# Autodesk Inventor assembly: Złożenie całości
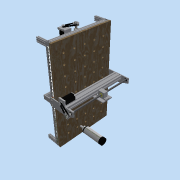
[picture p0: Inventor's stored thumbnail of the model, 180x180]
Saved by Autodesk Inventor 2018 (Build 220112000, 112)
## iProperties
Created: 2019-01-23
Part Number: Złożenie całości
Material: Ogólny
Document SubType Name: Assembly
Designer: Dawid
Author: Dawid
## Documents named in this file (38)
- E:\Frezarka_K2\INVENTOR\ZŁOŻENIA\Złożenie całości.iam
- E:\Frezarka_K2\INVENTOR\RAMA\Profil dolny długi.ipt
- E:\Frezarka_K2\INVENTOR\RAMA\Profil dolny krótki.ipt
- E:\Frezarka_K2\INVENTOR\RAMA\Profil dolny - noga.ipt
- E:\Frezarka_K2\INVENTOR\NAPĘD\Śruba trapezowa 16x4.ipt
- E:\Frezarka_K2\INVENTOR\NAPĘD\Łożysko w obudowie aluminiowej 10mm KP000.ipt
- C:\Users\Dawid\Documents\Inventor\Content Center Files\R2018\pl-PL\DIN 6926\DIN 6926 - M10 x 1,5.ipt
- E:\Frezarka_K2\INVENTOR\NAPĘD\Koło zębate 21 T5 28 2F.ipt
- E:\Frezarka_K2\INVENTOR\NAPĘD\Tuleja zaciskowo rozprężna RCK BK 80 8x15 Clampex.ipt
- C:\Users\Dawid\Documents\Inventor\Content Center Files\R2018\pl-PL\CNS 3932\CNS 3932 - M 4 x 0,7 x 6.ipt
- E:\Frezarka_K2\INVENTOR\NAPĘD\Silnik krokowy SM 60 100-4004AF - 4Nm.ipt
- E:\Frezarka_K2\INVENTOR\NAPĘD\Koło zębate 21 T5 14 2F.ipt
- E:\Frezarka_K2\INVENTOR\NAPĘD\Uchwyt silnika krokowego osi Y.ipt
- C:\Users\Dawid\Documents\Inventor\Content Center Files\R2018\pl-PL\CNS 3932\CNS 3932 - M 5 x 0,8 x 12.ipt
- C:\Users\Dawid\Documents\Inventor\Content Center Files\R2018\pl-PL\CNS 3932\CNS 3932 - M 5 x 0,8 x 10.ipt
- E:\Frezarka_K2\INVENTOR\NAPĘD\Nakrętka trapezowa kołnierzowa JFRM-2835TR16x4.ipt
- E:\Frezarka_K2\INVENTOR\NAPĘD\Obudowa nakrętki trapezowej fi 16.ipt
- E:\Frezarka_K2\INVENTOR\RAMA\Profil dolny posuwu osi Y.ipt
- E:\Frezarka_K2\INVENTOR\NAPĘD\Prowadnica liniowa MGN9R 900mm.ipt
- E:\Frezarka_K2\INVENTOR\NAPĘD\Wózek MGN9C.ipt
- C:\Users\Dawid\Documents\Inventor\Content Center Files\R2018\pl-PL\CNS 3932\CNS 3932 - M 3 x 0,5 x 5.ipt
- E:\Frezarka_K2\INVENTOR\WRZECIONA\Wrzeciono Elektrowrzeciono CNC 0.8kw.ipt
- E:\Frezarka_K2\INVENTOR\RAMA\Profil aluminiowy alutec K&K 104080.ipt
- E:\Frezarka_K2\INVENTOR\RAMA\Sklejka stołu.ipt
- E:\Frezarka_K2\INVENTOR\NAPĘD\Prowadnica liniowa typu MGN12H 600mm.ipt
- E:\Frezarka_K2\INVENTOR\NAPĘD\Wózek MGN12H.ipt
- E:\Frezarka_K2\INVENTOR\NAPĘD\Wspornik pionowy osi Z.ipt
- E:\Frezarka_K2\INVENTOR\NAPĘD\Łożysko kulowe jednorzędowe 6200 2RS.ipt
- E:\Frezarka_K2\INVENTOR\NAPĘD\Wspornik pionowy osi Y - lewa strona.ipt
- E:\Frezarka_K2\INVENTOR\NAPĘD\Wspornik pionowy osi Y - prawa strona.ipt
- E:\Frezarka_K2\INVENTOR\NAPĘD\Wspornik łożyska osi Y - prawa strona.ipt
- E:\Frezarka_K2\INVENTOR\NAPĘD\Łożysko kulowe jednorzędowe 3200 2RS.ipt
- E:\Frezarka_K2\INVENTOR\NAPĘD\Śruba trapezowa 16x4 - oś X.ipt
- C:\Users\Dawid\Documents\Inventor\Content Center Files\R2018\pl-PL\CNS 3932\CNS 3932 - M 3 x 0,5 x 14.ipt
- E:\Frezarka_K2\INVENTOR\NAPĘD\Uchwyt silnika krokowego osi X.ipt
- C:\Users\Dawid\Documents\Inventor\Content Center Files\R2018\pl-PL\CNS 3932\CNS 3932 - M 8 x 1,25 x 14.ipt
- E:\Frezarka_K2\INVENTOR\NAPĘD\Pas zębaty 10 T5-295.ipt
- C:\Users\Dawid\Documents\Inventor\Content Center Files\R2018\pl-PL\CNS 3932\CNS 3932 - M 4 x 0,7 x 16.ipt
## Components (206 placed, 37 different names)
1. Profil dolny długi:1 — Zestawiający:1, Zestawiający:4, Równoległy:19, Równoległy:20, Zestawiający:40, Równoległy:28, Równoległy:29, Zestawiający:41, Równoległy:30, Równoległy:31, Zestawiający:44, Równoległy:36, Równoległy:43, Równoległy:44, Równoległy:45, Zestawiający:65, Równoległy:53
2. Profil dolny krótki:1 — Zestawiający:1, Zestawiający:2, Równoległy:23, Równoległy:24, Zestawiający:38
3. Profil dolny długi:2 — Zestawiający:2, Zestawiający:5, Zestawiający:6, Równoległy:21, Równoległy:22, Równoległy:23, Równoległy:24, Zestawiający:39, Równoległy:26, Równoległy:27, Zestawiający:42, Równoległy:32, Równoległy:33, Zestawiający:45, Równoległy:38, Zestawiający:135
4. Profil dolny krótki:2 — Równoległy:19, Równoległy:20, Równoległy:21, Równoległy:22, Zestawiający:34, Równoległy:25, Zestawiający:36, Zestawiający:37, Równoległy:37, Równoległy:39, Równoległy:52, Zestawiający:135
5. Profil dolny - noga:1 — Zestawiający:5, Zestawiający:42, Równoległy:32, Równoległy:33
6. Profil dolny - noga:2 — Zestawiający:6, Zestawiający:39, Równoległy:26, Równoległy:27
7. Profil dolny - noga:3 — Zestawiający:41, Równoległy:30, Równoległy:31
8. Profil dolny - noga:4 — Zestawiający:4, Zestawiający:40, Równoległy:28, Równoległy:29, Zestawiający:64
9. Śruba trapezowa 16x4:1 — Zestawiający:8, Zestawiający:9, Zestawiający:10, Zestawiający:11, Zestawiający:12, Zestawiający:18, Zestawiający:19, Zestawiający:31
10. Łożysko w obudowie aluminiowej 10mm KP000:1 — Zestawiający:8, Zestawiający:9, Zestawiający:13, Zestawiający:34, Równoległy:25, Zestawiający:64
11. Łożysko w obudowie aluminiowej 10mm KP000:2 — Zestawiający:10, Zestawiający:11, Zestawiający:38
12. DIN 6926 - zastąpiona przez DIN EN 1663/1666 M10:1 — Zestawiający:12, Zestawiający:13
13. Koło zębate 21 T5 28 2F:1 — Zestawiający:16, Zestawiający:17, Zestawiający:136
14. Tuleja zaciskowo rozprężna RCK BK 80 8x15 Clampex:1 — Zestawiający:16, Zestawiający:17, Zestawiający:18, Zestawiający:19, Wstaw:1, Wstaw:2, Wstaw:3, Wstaw:4, Wstaw:5, Wstaw:6
15. CNS 3932 M 4 x 6:1 — Wstaw:1
16. CNS 3932 M 4 x 6:2 — Wstaw:2
17. CNS 3932 M 4 x 6:3 — Wstaw:3
18. CNS 3932 M 4 x 6:4 — Wstaw:4
19. CNS 3932 M 4 x 6:5 — Wstaw:5
20. CNS 3932 M 4 x 6:6 — Wstaw:6
21. Silnik krokowy SM 60 100-4004AF - 4Nm:1 — Zestawiający:21, Zestawiający:22, Zestawiający:23, Zestawiający:24, Zestawiający:25, Wstaw:7, Wstaw:8, Wstaw:9, Wstaw:10
22. Koło zębate 21 T5 14 2F:1 — Zestawiający:21, Zestawiający:22, Zestawiający:137, Zestawiający:138
23. Uchwyt silnika krokowego osi Y:1 — Zestawiający:23, Zestawiający:24, Zestawiający:25, Wstaw:11, Wstaw:12, Wstaw:13, Wstaw:14, Zestawiający:36, Zestawiający:37
24. CNS 3932 M 5 x 12:9 — Wstaw:7
25. CNS 3932 M 5 x 12:2 — Wstaw:8
26. CNS 3932 M 5 x 12:3 — Wstaw:9
27. CNS 3932 M 5 x 12:4 — Wstaw:10
28. CNS 3932 M 5 x 10:1 — Wstaw:11
29. CNS 3932 M 5 x 10:2 — Wstaw:12
30. CNS 3932 M 5 x 10:3 — Wstaw:13
31. CNS 3932 M 5 x 10:4 — Wstaw:14
32. Nakrętka trapezowa kołnierzowa JFRM-2835TR16x4:1 — Zestawiający:31, Zestawiający:112, Zestawiający:113, Wstaw:117, Wstaw:118, Wstaw:119, Wstaw:120, Wstaw:121, Wstaw:122
33. Obudowa nakrętki trapezowej fi 16:1 — Zestawiający:43, Równoległy:34, Wstaw:53, Wstaw:54, Wstaw:55, Wstaw:56, Zestawiający:112, Zestawiający:113
34. Profil dolny posuwu osi Y:1 — Zestawiający:43, Równoległy:34, Równoległy:40, Zestawiający:77, Równoległy:57, Równoległy:58, Zestawiający:79, Równoległy:60, Równoległy:61
35. Prowadnica liniowa MGN9R 900mm:1 — Zestawiający:44, Równoległy:36, Równoległy:37, Zestawiający:50, Zestawiający:51, Zestawiający:52, Zestawiający:53, Wstaw:34, Wstaw:35, Wstaw:36, Wstaw:37, Wstaw:38, Wstaw:39, Wstaw:40, Wstaw:41, Wstaw:42, Wstaw:43, Wstaw:44, Wstaw:45, Wstaw:46, Wstaw:47, Wstaw:48, Wstaw:49, Wstaw:50, Wstaw:51, Wstaw:52
36. Prowadnica liniowa MGN9R 900mm:2 — Zestawiający:45, Równoległy:38, Równoległy:39, Zestawiający:46, Zestawiający:47, Zestawiający:48, Zestawiający:49, Zestawiający:57, Wstaw:15, Wstaw:16, Wstaw:17, Wstaw:18, Wstaw:19, Wstaw:20, Wstaw:21, Wstaw:22, Wstaw:23, Wstaw:24, Wstaw:25, Wstaw:26, Wstaw:27, Wstaw:28, Wstaw:29, Wstaw:30, Wstaw:31, Wstaw:32, Wstaw:33
37. Wózek MGN9C:1 — Zestawiający:46, Zestawiający:47, Zestawiający:80
38. Wózek MGN9C:2 — Zestawiający:48, Zestawiający:49, Zestawiający:57, Zestawiający:81
39. Wózek MGN9C:3 — Zestawiający:50, Zestawiający:51, Zestawiający:82
40. Wózek MGN9C:4 — Zestawiający:52, Zestawiający:53, Równoległy:40, Zestawiający:83
41. CNS 3932 M 3 x 5:1 — Wstaw:15
42. CNS 3932 M 3 x 5:2 — Wstaw:16
43. CNS 3932 M 3 x 5:3 — Wstaw:17
44. CNS 3932 M 3 x 5:4 — Wstaw:18
45. CNS 3932 M 3 x 5:5 — Wstaw:19
46. CNS 3932 M 3 x 5:6 — Wstaw:20
47. CNS 3932 M 3 x 5:7 — Wstaw:21
48. CNS 3932 M 3 x 5:8 — Wstaw:22
49. CNS 3932 M 3 x 5:9 — Wstaw:23
50. CNS 3932 M 3 x 5:10 — Wstaw:24
51. CNS 3932 M 3 x 5:11 — Wstaw:25
52. CNS 3932 M 3 x 5:12 — Wstaw:26
53. CNS 3932 M 3 x 5:13 — Wstaw:27
54. CNS 3932 M 3 x 5:14 — Wstaw:28
55. CNS 3932 M 3 x 5:15 — Wstaw:29
56. CNS 3932 M 3 x 5:16 — Wstaw:30
57. CNS 3932 M 3 x 5:17 — Wstaw:31
58. CNS 3932 M 3 x 5:18 — Wstaw:32
59. CNS 3932 M 3 x 5:19 — Wstaw:33
60. CNS 3932 M 3 x 5:20 — Wstaw:34
61. CNS 3932 M 3 x 5:21 — Wstaw:35
62. CNS 3932 M 3 x 5:22 — Wstaw:36
63. CNS 3932 M 3 x 5:23 — Wstaw:37
64. CNS 3932 M 3 x 5:24 — Wstaw:38
65. CNS 3932 M 3 x 5:25 — Wstaw:39
66. CNS 3932 M 3 x 5:26 — Wstaw:40
67. CNS 3932 M 3 x 5:27 — Wstaw:41
68. CNS 3932 M 3 x 5:28 — Wstaw:42
69. CNS 3932 M 3 x 5:29 — Wstaw:43
70. CNS 3932 M 3 x 5:30 — Wstaw:44
71. CNS 3932 M 3 x 5:31 — Wstaw:45
72. CNS 3932 M 3 x 5:32 — Wstaw:46
73. CNS 3932 M 3 x 5:33 — Wstaw:47
74. CNS 3932 M 3 x 5:34 — Wstaw:48
75. CNS 3932 M 3 x 5:35 — Wstaw:49
76. CNS 3932 M 3 x 5:36 — Wstaw:50
77. CNS 3932 M 3 x 5:37 — Wstaw:51
78. CNS 3932 M 3 x 5:38 — Wstaw:52
79. Wrzeciono Elektrowrzeciono CNC 0.8kw:1 — Zestawiający:94
80. CNS 3932 M 5 x 10:5 — Wstaw:53
81. CNS 3932 M 5 x 10:6 — Wstaw:54
82. CNS 3932 M 5 x 10:7 — Wstaw:55
83. CNS 3932 M 5 x 10:8 — Wstaw:56
84. Profil aluminiowy alutec K&K 104080:1 — Zestawiający:66, Równoległy:54, Zestawiający:68, Równoległy:55, Równoległy:63, Równoległy:64, Zestawiający:84, Równoległy:65, Równoległy:66
85. Sklejka stołu:1 — Zestawiający:65, Równoległy:52, Równoległy:53, Zestawiający:94
86. Prowadnica liniowa typu MGN12H 600mm:1 — Zestawiający:68, Równoległy:55, Wstaw:80, Wstaw:81, Wstaw:82, Wstaw:83, Wstaw:84, Wstaw:85, Wstaw:86, Wstaw:87, Wstaw:88, Wstaw:89, Wstaw:90, Wstaw:91, Wstaw:92, Wstaw:93, Wstaw:94, Wstaw:95, Wstaw:96, Wstaw:97, Wstaw:98, Wstaw:99, Wstaw:100, Wstaw:101, Wstaw:102, Zestawiający:72, Zestawiający:73, Równoległy:64
87. Prowadnica liniowa typu MGN12H 600mm:2 — Zestawiający:66, Równoległy:54, Wstaw:57, Wstaw:58, Wstaw:59, Wstaw:60, Wstaw:61, Wstaw:62, Wstaw:63, Wstaw:64, Wstaw:65, Wstaw:66, Wstaw:67, Wstaw:68, Wstaw:69, Wstaw:70, Wstaw:71, Wstaw:72, Wstaw:73, Wstaw:74, Wstaw:75, Wstaw:76, Wstaw:77, Wstaw:78, Wstaw:79, Zestawiający:70, Zestawiający:71, Równoległy:63
88. CNS 3932 M 3 x 5:39 — Wstaw:57
89. CNS 3932 M 3 x 5:40 — Wstaw:58
90. CNS 3932 M 3 x 5:41 — Wstaw:59
91. CNS 3932 M 3 x 5:42 — Wstaw:60
92. CNS 3932 M 3 x 5:43 — Wstaw:61
93. CNS 3932 M 3 x 5:44 — Wstaw:62
94. CNS 3932 M 3 x 5:45 — Wstaw:63
95. CNS 3932 M 3 x 5:46 — Wstaw:64
96. CNS 3932 M 3 x 5:47 — Wstaw:65
97. CNS 3932 M 3 x 5:48 — Wstaw:66
98. CNS 3932 M 3 x 5:49 — Wstaw:67
99. CNS 3932 M 3 x 5:50 — Wstaw:68
100. CNS 3932 M 3 x 5:51 — Wstaw:69
101. CNS 3932 M 3 x 5:52 — Wstaw:70
102. CNS 3932 M 3 x 5:53 — Wstaw:71
103. CNS 3932 M 3 x 5:54 — Wstaw:72
104. CNS 3932 M 3 x 5:55 — Wstaw:73
105. CNS 3932 M 3 x 5:56 — Wstaw:74
106. CNS 3932 M 3 x 5:57 — Wstaw:75
107. CNS 3932 M 3 x 5:58 — Wstaw:76
108. CNS 3932 M 3 x 5:59 — Wstaw:77
109. CNS 3932 M 3 x 5:60 — Wstaw:78
110. CNS 3932 M 3 x 5:61 — Wstaw:79
111. CNS 3932 M 3 x 5:62 — Wstaw:80
112. CNS 3932 M 3 x 5:63 — Wstaw:81
113. CNS 3932 M 3 x 5:64 — Wstaw:82
114. CNS 3932 M 3 x 5:65 — Wstaw:83
115. CNS 3932 M 3 x 5:66 — Wstaw:84
116. CNS 3932 M 3 x 5:67 — Wstaw:85
117. CNS 3932 M 3 x 5:68 — Wstaw:86
118. CNS 3932 M 3 x 5:69 — Wstaw:87
119. CNS 3932 M 3 x 5:70 — Wstaw:88
120. CNS 3932 M 3 x 5:71 — Wstaw:89
121. CNS 3932 M 3 x 5:72 — Wstaw:90
122. CNS 3932 M 3 x 5:73 — Wstaw:91
123. CNS 3932 M 3 x 5:74 — Wstaw:92
124. CNS 3932 M 3 x 5:75 — Wstaw:93
125. CNS 3932 M 3 x 5:76 — Wstaw:94
126. CNS 3932 M 3 x 5:77 — Wstaw:95
127. CNS 3932 M 3 x 5:78 — Wstaw:96
128. CNS 3932 M 3 x 5:79 — Wstaw:97
129. CNS 3932 M 3 x 5:80 — Wstaw:98
130. CNS 3932 M 3 x 5:81 — Wstaw:99
131. CNS 3932 M 3 x 5:82 — Wstaw:100
132. CNS 3932 M 3 x 5:83 — Wstaw:101
133. CNS 3932 M 3 x 5:84 — Wstaw:102
134. Wózek MGN12H:1 — Zestawiający:70, Zestawiający:71, Zestawiający:74, Równoległy:56, Zestawiający:76
135. Wózek MGN12H:2 — Zestawiający:72, Zestawiający:73, Zestawiający:75, Równoległy:56
136. Wspornik pionowy osi Z:1 — Wstaw:103, Wstaw:104, Wstaw:105, Wstaw:106, Wstaw:107, Wstaw:108, Wstaw:109, Wstaw:110, Zestawiający:74, Zestawiający:75, Zestawiający:76, Zestawiający:106, Zestawiający:107, Zestawiający:108
137. CNS 3932 M 3 x 5:85 — Wstaw:103
138. CNS 3932 M 3 x 5:86 — Wstaw:104
139. CNS 3932 M 3 x 5:87 — Wstaw:105
140. CNS 3932 M 3 x 5:88 — Wstaw:106
141. CNS 3932 M 3 x 5:89 — Wstaw:107
142. CNS 3932 M 3 x 5:90 — Wstaw:108
143. CNS 3932 M 3 x 5:91 — Wstaw:109
144. CNS 3932 M 3 x 5:92 — Wstaw:110
145. Łożysko kulowe jednorzędowe 6200 2RS:1 — Zestawiający:78, Równoległy:59
146. Wspornik pionowy osi Y - lewa strona:1 — Zestawiający:77, Równoległy:57, Równoległy:58, Zestawiający:78, Równoległy:59, Zestawiający:80, Zestawiający:81, Wstaw:133, Wstaw:134
147. Wspornik pionowy osi Y - prawa strona:1 — Zestawiający:79, Równoległy:60, Równoległy:61, Zestawiający:82, Zestawiający:83, Zestawiający:84, Równoległy:65, Równoległy:66, Zestawiający:96, Równoległy:67, Zestawiający:97, Równoległy:68, Równoległy:69, Zestawiający:120, Wstaw:135, Wstaw:136, Wstaw:145, Wstaw:146, Wstaw:147, Wstaw:148, Wstaw:149, Wstaw:150, Wstaw:151, Wstaw:152, Zestawiający:139, Zestawiający:141, Zestawiający:143, Zestawiający:145
148. Łożysko kulowe jednorzędowe 3200 2RS:1 — Zestawiający:87, Zestawiający:88, Zestawiający:90, Zestawiający:96, Równoległy:69
149. Silnik krokowy SM 60 100-4004AF - 4Nm:2 — Zestawiający:118, Zestawiający:119, Zestawiający:120, Zestawiający:123, Zestawiający:124, Zestawiający:125, Wstaw:153, Wstaw:154, Wstaw:155, Wstaw:156
150. Śruba trapezowa 16x4 - oś X:1 — Zestawiający:87, Zestawiający:88, Zestawiający:89, Zestawiający:116, Zestawiający:117
151. DIN 6926 - zastąpiona przez DIN EN 1663/1666 M10:2 — Zestawiający:89, Zestawiający:90
152. Nakrętka trapezowa kołnierzowa JFRM-2835TR16x4:2 — Zestawiający:109, Zestawiający:110, Zestawiający:111, Wstaw:111, Wstaw:112, Wstaw:113, Wstaw:114, Wstaw:115, Wstaw:116
153. Obudowa nakrętki trapezowej fi 16:2 — Zestawiający:106, Zestawiający:107, Zestawiający:108, Zestawiający:109, Zestawiający:110, Zestawiający:111, Wstaw:123, Wstaw:124, Wstaw:125, Wstaw:126
154. Wspornik łożyska osi Y - prawa strona:1 — Równoległy:67, Zestawiający:97, Równoległy:68, Zestawiający:98, Zestawiający:99, Zestawiający:100, Zestawiający:101, Zestawiający:102, Zestawiający:103, Zestawiający:104, Zestawiający:105
155. CNS 3932 M 3 x 14:2 — Zestawiający:98, Zestawiający:99
156. CNS 3932 M 3 x 14:3 — Zestawiający:100, Zestawiający:101
157. CNS 3932 M 3 x 14:1 — Zestawiający:102, Zestawiający:103
158. CNS 3932 M 3 x 14:4 — Zestawiający:104, Zestawiający:105
159. CNS 3932 M 5 x 10:9 — Wstaw:111
160. CNS 3932 M 5 x 10:10 — Wstaw:112
161. CNS 3932 M 5 x 10:11 — Wstaw:113
162. CNS 3932 M 5 x 10:12 — Wstaw:114
163. CNS 3932 M 5 x 10:13 — Wstaw:115
164. CNS 3932 M 5 x 10:14 — Wstaw:116
165. CNS 3932 M 5 x 10:15 — Wstaw:117
166. CNS 3932 M 5 x 10:16 — Wstaw:118
167. CNS 3932 M 5 x 10:17 — Wstaw:119
168. CNS 3932 M 5 x 10:18 — Wstaw:120
169. CNS 3932 M 5 x 10:19 — Wstaw:121
170. CNS 3932 M 5 x 10:20 — Wstaw:122
171. CNS 3932 M 5 x 12:5 — Wstaw:123
172. CNS 3932 M 5 x 12:8 — Wstaw:124
173. CNS 3932 M 5 x 12:6 — Wstaw:125
174. CNS 3932 M 5 x 12:7 — Wstaw:126
175. Koło zębate 21 T5 28 2F:2 — Zestawiający:114, Zestawiający:115, Równoległy:70, Zestawiający:129
176. Tuleja zaciskowo rozprężna RCK BK 80 8x15 Clampex:2 — Zestawiający:114, Zestawiający:115, Zestawiający:116, Wstaw:127, Wstaw:128, Wstaw:129, Wstaw:130, Wstaw:131, Wstaw:132, Zestawiający:117
177. CNS 3932 M 4 x 6:7 — Wstaw:127
178. CNS 3932 M 4 x 6:8 — Wstaw:128
179. CNS 3932 M 4 x 6:9 — Wstaw:129
180. CNS 3932 M 4 x 6:10 — Wstaw:130
181. CNS 3932 M 4 x 6:11 — Wstaw:131
182. CNS 3932 M 4 x 6:12 — Wstaw:132
183. Koło zębate 21 T5 14 2F:2 — Zestawiający:118, Zestawiający:119, Równoległy:70, Zestawiający:130, Zestawiający:131
184. Uchwyt silnika krokowego osi X:1 — Zestawiający:123, Zestawiający:124, Zestawiający:125, Zestawiający:140, Zestawiający:142, Zestawiający:144, Zestawiający:146
185. CNS 3932 M 8 x 14:1 — Wstaw:133
186. CNS 3932 M 8 x 14:2 — Wstaw:134
187. CNS 3932 M 8 x 14:3 — Wstaw:135
188. CNS 3932 M 8 x 14:4 — Wstaw:136
189. Pas zębaty 10 T5-295:1 — Zestawiający:129, Zestawiający:130, Zestawiający:131
190. Pas zębaty 10 T5-295:2 — Zestawiający:136, Zestawiający:137, Zestawiający:138
191. CNS 3932 M 4 x 16:1 — Zestawiający:139, Zestawiający:140
192. CNS 3932 M 4 x 16:4 — Zestawiający:145, Zestawiający:146
193. CNS 3932 M 4 x 16:2 — Zestawiający:141, Zestawiający:142
194. CNS 3932 M 4 x 16:3 — Zestawiający:143, Zestawiający:144
195. CNS 3932 M 4 x 6:21 — Wstaw:145
196. CNS 3932 M 4 x 6:22 — Wstaw:146
197. CNS 3932 M 4 x 6:23 — Wstaw:147
198. CNS 3932 M 4 x 6:24 — Wstaw:148
199. CNS 3932 M 4 x 6:25 — Wstaw:149
200. CNS 3932 M 4 x 6:26 — Wstaw:150
201. CNS 3932 M 4 x 6:27 — Wstaw:151
202. CNS 3932 M 4 x 6:28 — Wstaw:152
203. CNS 3932 M 5 x 12:10 — Wstaw:153
204. CNS 3932 M 5 x 12:11 — Wstaw:154
205. CNS 3932 M 5 x 12:12 — Wstaw:155
206. CNS 3932 M 5 x 12:13 — Wstaw:156
## Relationships (298: Insert 148, Mate 108, Flush 42)
- Zestawiający:1 [Mate]: Profil dolny długi:1 ↔ Profil dolny krótki:1
- Zestawiający:2 [Mate]: Profil dolny krótki:1 ↔ Profil dolny długi:2
- Zestawiający:4 [Mate]: Profil dolny długi:1 ↔ Profil dolny - noga:4
- Zestawiający:5 [Mate]: Profil dolny długi:2 ↔ Profil dolny - noga:1
- Zestawiający:6 [Mate]: Profil dolny długi:2 ↔ Profil dolny - noga:2
- Zestawiający:8 [Mate]: Śruba trapezowa 16x4:1 ↔ Łożysko w obudowie aluminiowej 10mm KP000:1
- Zestawiający:9 [Mate]: Śruba trapezowa 16x4:1 ↔ Łożysko w obudowie aluminiowej 10mm KP000:1
- Zestawiający:10 [Mate]: Śruba trapezowa 16x4:1 ↔ Łożysko w obudowie aluminiowej 10mm KP000:2
- Zestawiający:11 [Mate] (2 mm): Śruba trapezowa 16x4:1 ↔ Łożysko w obudowie aluminiowej 10mm KP000:2
- Zestawiający:12 [Mate]: Śruba trapezowa 16x4:1 ↔ DIN 6926 - zastąpiona przez DIN EN 1663/1666 M10:1
- Zestawiający:13 [Mate]: Łożysko w obudowie aluminiowej 10mm KP000:1 ↔ DIN 6926 - zastąpiona przez DIN EN 1663/1666 M10:1
- Zestawiający:16 [Mate]: Koło zębate 21 T5 28 2F:1 ↔ Tuleja zaciskowo rozprężna RCK BK 80 8x15 Clampex:1
- Zestawiający:17 [Mate]: Koło zębate 21 T5 28 2F:1 ↔ Tuleja zaciskowo rozprężna RCK BK 80 8x15 Clampex:1
- Zestawiający:18 [Mate]: Śruba trapezowa 16x4:1 ↔ Tuleja zaciskowo rozprężna RCK BK 80 8x15 Clampex:1
- Zestawiający:19 [Mate] (2 mm): Śruba trapezowa 16x4:1 ↔ Tuleja zaciskowo rozprężna RCK BK 80 8x15 Clampex:1
- Wstaw:1 [Insert]: Tuleja zaciskowo rozprężna RCK BK 80 8x15 Clampex:1 ↔ CNS 3932 M 4 x 6:1
- Wstaw:2 [Insert]: Tuleja zaciskowo rozprężna RCK BK 80 8x15 Clampex:1 ↔ CNS 3932 M 4 x 6:2
- Wstaw:3 [Insert]: Tuleja zaciskowo rozprężna RCK BK 80 8x15 Clampex:1 ↔ CNS 3932 M 4 x 6:3
- Wstaw:4 [Insert]: Tuleja zaciskowo rozprężna RCK BK 80 8x15 Clampex:1 ↔ CNS 3932 M 4 x 6:4
- Wstaw:5 [Insert]: Tuleja zaciskowo rozprężna RCK BK 80 8x15 Clampex:1 ↔ CNS 3932 M 4 x 6:5
- Wstaw:6 [Insert]: Tuleja zaciskowo rozprężna RCK BK 80 8x15 Clampex:1 ↔ CNS 3932 M 4 x 6:6
- Zestawiający:21 [Mate]: Silnik krokowy SM 60 100-4004AF - 4Nm:1 ↔ Koło zębate 21 T5 14 2F:1
- Zestawiający:22 [Mate] (1 mm): Silnik krokowy SM 60 100-4004AF - 4Nm:1 ↔ Koło zębate 21 T5 14 2F:1
- Zestawiający:23 [Mate]: Silnik krokowy SM 60 100-4004AF - 4Nm:1 ↔ Uchwyt silnika krokowego osi Y:1
- Zestawiający:24 [Mate]: Silnik krokowy SM 60 100-4004AF - 4Nm:1 ↔ Uchwyt silnika krokowego osi Y:1
- Zestawiający:25 [Mate]: Silnik krokowy SM 60 100-4004AF - 4Nm:1 ↔ Uchwyt silnika krokowego osi Y:1
- Wstaw:7 [Insert]: Silnik krokowy SM 60 100-4004AF - 4Nm:1 ↔ CNS 3932 M 5 x 12:9
- Wstaw:8 [Insert]: Silnik krokowy SM 60 100-4004AF - 4Nm:1 ↔ CNS 3932 M 5 x 12:2
- Wstaw:9 [Insert]: Silnik krokowy SM 60 100-4004AF - 4Nm:1 ↔ CNS 3932 M 5 x 12:3
- Wstaw:10 [Insert]: Silnik krokowy SM 60 100-4004AF - 4Nm:1 ↔ CNS 3932 M 5 x 12:4
- Wstaw:11 [Insert]: Uchwyt silnika krokowego osi Y:1 ↔ CNS 3932 M 5 x 10:1
- Wstaw:12 [Insert]: Uchwyt silnika krokowego osi Y:1 ↔ CNS 3932 M 5 x 10:2
- Wstaw:13 [Insert]: Uchwyt silnika krokowego osi Y:1 ↔ CNS 3932 M 5 x 10:3
- Wstaw:14 [Insert]: Uchwyt silnika krokowego osi Y:1 ↔ CNS 3932 M 5 x 10:4
- Zestawiający:31 [Mate]: Śruba trapezowa 16x4:1 ↔ Nakrętka trapezowa kołnierzowa JFRM-2835TR16x4:1
- Równoległy:19 [Flush]: Profil dolny długi:1 ↔ Profil dolny krótki:2
- Równoległy:20 [Flush]: Profil dolny długi:1 ↔ Profil dolny krótki:2
- Równoległy:21 [Flush]: Profil dolny długi:2 ↔ Profil dolny krótki:2
- Równoległy:22 [Flush]: Profil dolny długi:2 ↔ Profil dolny krótki:2
- Równoległy:23 [Flush]: Profil dolny krótki:1 ↔ Profil dolny długi:2
- Równoległy:24 [Flush]: Profil dolny krótki:1 ↔ Profil dolny długi:2
- Zestawiający:34 [Mate]: Profil dolny krótki:2 ↔ Łożysko w obudowie aluminiowej 10mm KP000:1
- Równoległy:25 [Flush] (2 mm): Profil dolny krótki:2 ↔ Łożysko w obudowie aluminiowej 10mm KP000:1
- Zestawiający:36 [Mate]: Profil dolny krótki:2 ↔ Uchwyt silnika krokowego osi Y:1
- Zestawiający:37 [Mate]: Profil dolny krótki:2 ↔ Uchwyt silnika krokowego osi Y:1
- Zestawiający:38 [Mate]: Profil dolny krótki:1 ↔ Łożysko w obudowie aluminiowej 10mm KP000:2
- Zestawiający:39 [Mate]: Profil dolny długi:2 ↔ Profil dolny - noga:2
- Równoległy:26 [Flush]: Profil dolny długi:2 ↔ Profil dolny - noga:2
- Równoległy:27 [Flush]: Profil dolny długi:2 ↔ Profil dolny - noga:2
- Zestawiający:40 [Mate]: Profil dolny długi:1 ↔ Profil dolny - noga:4
- Równoległy:28 [Flush]: Profil dolny długi:1 ↔ Profil dolny - noga:4
- Równoległy:29 [Flush]: Profil dolny długi:1 ↔ Profil dolny - noga:4
- Zestawiający:41 [Mate]: Profil dolny długi:1 ↔ Profil dolny - noga:3
- Równoległy:30 [Flush]: Profil dolny długi:1 ↔ Profil dolny - noga:3
- Równoległy:31 [Flush]: Profil dolny długi:1 ↔ Profil dolny - noga:3
- Zestawiający:42 [Mate]: Profil dolny długi:2 ↔ Profil dolny - noga:1
- Równoległy:32 [Flush]: Profil dolny długi:2 ↔ Profil dolny - noga:1
- Równoległy:33 [Flush]: Profil dolny długi:2 ↔ Profil dolny - noga:1
- Zestawiający:43 [Mate]: Obudowa nakrętki trapezowej fi 16:1 ↔ Profil dolny posuwu osi Y:1
- Równoległy:34 [Flush]: Obudowa nakrętki trapezowej fi 16:1 ↔ Profil dolny posuwu osi Y:1
- Zestawiający:44 [Mate]: Profil dolny długi:1 ↔ Prowadnica liniowa MGN9R 900mm:1
- Równoległy:36 [Flush] (25.5 mm): Profil dolny długi:1 ↔ Prowadnica liniowa MGN9R 900mm:1
- Równoległy:37 [Flush] (25 mm): Profil dolny krótki:2 ↔ Prowadnica liniowa MGN9R 900mm:1
- Zestawiający:45 [Mate]: Profil dolny długi:2 ↔ Prowadnica liniowa MGN9R 900mm:2
- Równoległy:38 [Flush] (25.5 mm): Profil dolny długi:2 ↔ Prowadnica liniowa MGN9R 900mm:2
- Równoległy:39 [Flush] (25 mm): Profil dolny krótki:2 ↔ Prowadnica liniowa MGN9R 900mm:2
- Zestawiający:46 [Mate]: Prowadnica liniowa MGN9R 900mm:2 ↔ Wózek MGN9C:1
- Zestawiający:47 [Mate]: Prowadnica liniowa MGN9R 900mm:2 ↔ Wózek MGN9C:1
- Zestawiający:48 [Mate]: Prowadnica liniowa MGN9R 900mm:2 ↔ Wózek MGN9C:2
- Zestawiający:49 [Mate]: Prowadnica liniowa MGN9R 900mm:2 ↔ Wózek MGN9C:2
- Zestawiający:50 [Mate]: Prowadnica liniowa MGN9R 900mm:1 ↔ Wózek MGN9C:3
- Zestawiający:51 [Mate]: Prowadnica liniowa MGN9R 900mm:1 ↔ Wózek MGN9C:3
- Zestawiający:52 [Mate]: Prowadnica liniowa MGN9R 900mm:1 ↔ Wózek MGN9C:4
- Zestawiający:53 [Mate]: Prowadnica liniowa MGN9R 900mm:1 ↔ Wózek MGN9C:4
- Równoległy:40 [Flush]: Profil dolny posuwu osi Y:1 ↔ Wózek MGN9C:4
- Równoległy:43 [Flush]: Profil dolny długi:1
- Równoległy:44 [Flush]: Profil dolny długi:1
- Równoległy:45 [Flush]: Profil dolny długi:1
- Zestawiający:57 [Mate]: Prowadnica liniowa MGN9R 900mm:2 ↔ Wózek MGN9C:2
- Wstaw:15 [Insert]: Prowadnica liniowa MGN9R 900mm:2 ↔ CNS 3932 M 3 x 5:1
- Wstaw:16 [Insert]: Prowadnica liniowa MGN9R 900mm:2 ↔ CNS 3932 M 3 x 5:2
- Wstaw:17 [Insert]: Prowadnica liniowa MGN9R 900mm:2 ↔ CNS 3932 M 3 x 5:3
- Wstaw:18 [Insert]: Prowadnica liniowa MGN9R 900mm:2 ↔ CNS 3932 M 3 x 5:4
- Wstaw:19 [Insert]: Prowadnica liniowa MGN9R 900mm:2 ↔ CNS 3932 M 3 x 5:5
- Wstaw:20 [Insert]: Prowadnica liniowa MGN9R 900mm:2 ↔ CNS 3932 M 3 x 5:6
- Wstaw:21 [Insert]: Prowadnica liniowa MGN9R 900mm:2 ↔ CNS 3932 M 3 x 5:7
- Wstaw:22 [Insert]: Prowadnica liniowa MGN9R 900mm:2 ↔ CNS 3932 M 3 x 5:8
- Wstaw:23 [Insert]: Prowadnica liniowa MGN9R 900mm:2 ↔ CNS 3932 M 3 x 5:9
- Wstaw:24 [Insert]: Prowadnica liniowa MGN9R 900mm:2 ↔ CNS 3932 M 3 x 5:10
- Wstaw:25 [Insert]: Prowadnica liniowa MGN9R 900mm:2 ↔ CNS 3932 M 3 x 5:11
- Wstaw:26 [Insert]: Prowadnica liniowa MGN9R 900mm:2 ↔ CNS 3932 M 3 x 5:12
- Wstaw:27 [Insert]: Prowadnica liniowa MGN9R 900mm:2 ↔ CNS 3932 M 3 x 5:13
- Wstaw:28 [Insert]: Prowadnica liniowa MGN9R 900mm:2 ↔ CNS 3932 M 3 x 5:14
- Wstaw:29 [Insert]: Prowadnica liniowa MGN9R 900mm:2 ↔ CNS 3932 M 3 x 5:15
- Wstaw:30 [Insert]: Prowadnica liniowa MGN9R 900mm:2 ↔ CNS 3932 M 3 x 5:16
- Wstaw:31 [Insert]: Prowadnica liniowa MGN9R 900mm:2 ↔ CNS 3932 M 3 x 5:17
- Wstaw:32 [Insert]: Prowadnica liniowa MGN9R 900mm:2 ↔ CNS 3932 M 3 x 5:18
- Wstaw:33 [Insert]: Prowadnica liniowa MGN9R 900mm:2 ↔ CNS 3932 M 3 x 5:19
- Wstaw:34 [Insert]: Prowadnica liniowa MGN9R 900mm:1 ↔ CNS 3932 M 3 x 5:20
- Wstaw:35 [Insert]: Prowadnica liniowa MGN9R 900mm:1 ↔ CNS 3932 M 3 x 5:21
- Wstaw:36 [Insert]: Prowadnica liniowa MGN9R 900mm:1 ↔ CNS 3932 M 3 x 5:22
- Wstaw:37 [Insert]: Prowadnica liniowa MGN9R 900mm:1 ↔ CNS 3932 M 3 x 5:23
- Wstaw:38 [Insert]: Prowadnica liniowa MGN9R 900mm:1 ↔ CNS 3932 M 3 x 5:24
- Wstaw:39 [Insert]: Prowadnica liniowa MGN9R 900mm:1 ↔ CNS 3932 M 3 x 5:25
- Wstaw:40 [Insert]: Prowadnica liniowa MGN9R 900mm:1 ↔ CNS 3932 M 3 x 5:26
- Wstaw:41 [Insert]: Prowadnica liniowa MGN9R 900mm:1 ↔ CNS 3932 M 3 x 5:27
- Wstaw:42 [Insert]: Prowadnica liniowa MGN9R 900mm:1 ↔ CNS 3932 M 3 x 5:28
- Wstaw:43 [Insert]: Prowadnica liniowa MGN9R 900mm:1 ↔ CNS 3932 M 3 x 5:29
- Wstaw:44 [Insert]: Prowadnica liniowa MGN9R 900mm:1 ↔ CNS 3932 M 3 x 5:30
- Wstaw:45 [Insert]: Prowadnica liniowa MGN9R 900mm:1 ↔ CNS 3932 M 3 x 5:31
- Wstaw:46 [Insert]: Prowadnica liniowa MGN9R 900mm:1 ↔ CNS 3932 M 3 x 5:32
- Wstaw:47 [Insert]: Prowadnica liniowa MGN9R 900mm:1 ↔ CNS 3932 M 3 x 5:33
- Wstaw:48 [Insert]: Prowadnica liniowa MGN9R 900mm:1 ↔ CNS 3932 M 3 x 5:34
- Wstaw:49 [Insert]: Prowadnica liniowa MGN9R 900mm:1 ↔ CNS 3932 M 3 x 5:35
- Wstaw:50 [Insert]: Prowadnica liniowa MGN9R 900mm:1 ↔ CNS 3932 M 3 x 5:36
- Wstaw:51 [Insert]: Prowadnica liniowa MGN9R 900mm:1 ↔ CNS 3932 M 3 x 5:37
- Wstaw:52 [Insert]: Prowadnica liniowa MGN9R 900mm:1 ↔ CNS 3932 M 3 x 5:38
- Wstaw:53 [Insert]: Obudowa nakrętki trapezowej fi 16:1 ↔ CNS 3932 M 5 x 10:5
- Wstaw:54 [Insert]: Obudowa nakrętki trapezowej fi 16:1 ↔ CNS 3932 M 5 x 10:6
- Wstaw:55 [Insert]: Obudowa nakrętki trapezowej fi 16:1 ↔ CNS 3932 M 5 x 10:7
- Wstaw:56 [Insert]: Obudowa nakrętki trapezowej fi 16:1 ↔ CNS 3932 M 5 x 10:8
- Zestawiający:64 [Mate] (236.5 mm): Profil dolny - noga:4 ↔ Łożysko w obudowie aluminiowej 10mm KP000:1
- Zestawiający:65 [Mate]: Profil dolny długi:1 ↔ Sklejka stołu:1
- Równoległy:52 [Flush]: Profil dolny krótki:2 ↔ Sklejka stołu:1
- Równoległy:53 [Flush]: Profil dolny długi:1 ↔ Sklejka stołu:1
- Zestawiający:66 [Mate]: Profil aluminiowy alutec K&K 104080:1 ↔ Prowadnica liniowa typu MGN12H 600mm:2
- Równoległy:54 [Flush] (14 mm): Profil aluminiowy alutec K&K 104080:1 ↔ Prowadnica liniowa typu MGN12H 600mm:2
- Zestawiający:68 [Mate]: Profil aluminiowy alutec K&K 104080:1 ↔ Prowadnica liniowa typu MGN12H 600mm:1
- Równoległy:55 [Flush] (14 mm): Profil aluminiowy alutec K&K 104080:1 ↔ Prowadnica liniowa typu MGN12H 600mm:1
- Wstaw:57 [Insert]: Prowadnica liniowa typu MGN12H 600mm:2 ↔ CNS 3932 M 3 x 5:39
- Wstaw:58 [Insert]: Prowadnica liniowa typu MGN12H 600mm:2 ↔ CNS 3932 M 3 x 5:40
- Wstaw:59 [Insert]: Prowadnica liniowa typu MGN12H 600mm:2 ↔ CNS 3932 M 3 x 5:41
- Wstaw:60 [Insert]: Prowadnica liniowa typu MGN12H 600mm:2 ↔ CNS 3932 M 3 x 5:42
- Wstaw:61 [Insert]: Prowadnica liniowa typu MGN12H 600mm:2 ↔ CNS 3932 M 3 x 5:43
- Wstaw:62 [Insert]: Prowadnica liniowa typu MGN12H 600mm:2 ↔ CNS 3932 M 3 x 5:44
- Wstaw:63 [Insert]: Prowadnica liniowa typu MGN12H 600mm:2 ↔ CNS 3932 M 3 x 5:45
- Wstaw:64 [Insert]: Prowadnica liniowa typu MGN12H 600mm:2 ↔ CNS 3932 M 3 x 5:46
- Wstaw:65 [Insert]: Prowadnica liniowa typu MGN12H 600mm:2 ↔ CNS 3932 M 3 x 5:47
- Wstaw:66 [Insert]: Prowadnica liniowa typu MGN12H 600mm:2 ↔ CNS 3932 M 3 x 5:48
- Wstaw:67 [Insert]: Prowadnica liniowa typu MGN12H 600mm:2 ↔ CNS 3932 M 3 x 5:49
- Wstaw:68 [Insert]: Prowadnica liniowa typu MGN12H 600mm:2 ↔ CNS 3932 M 3 x 5:50
- Wstaw:69 [Insert]: Prowadnica liniowa typu MGN12H 600mm:2 ↔ CNS 3932 M 3 x 5:51
- Wstaw:70 [Insert]: Prowadnica liniowa typu MGN12H 600mm:2 ↔ CNS 3932 M 3 x 5:52
- Wstaw:71 [Insert]: Prowadnica liniowa typu MGN12H 600mm:2 ↔ CNS 3932 M 3 x 5:53
- Wstaw:72 [Insert]: Prowadnica liniowa typu MGN12H 600mm:2 ↔ CNS 3932 M 3 x 5:54
- Wstaw:73 [Insert]: Prowadnica liniowa typu MGN12H 600mm:2 ↔ CNS 3932 M 3 x 5:55
- Wstaw:74 [Insert]: Prowadnica liniowa typu MGN12H 600mm:2 ↔ CNS 3932 M 3 x 5:56
- Wstaw:75 [Insert]: Prowadnica liniowa typu MGN12H 600mm:2 ↔ CNS 3932 M 3 x 5:57
- Wstaw:76 [Insert]: Prowadnica liniowa typu MGN12H 600mm:2 ↔ CNS 3932 M 3 x 5:58
- Wstaw:77 [Insert]: Prowadnica liniowa typu MGN12H 600mm:2 ↔ CNS 3932 M 3 x 5:59
- Wstaw:78 [Insert]: Prowadnica liniowa typu MGN12H 600mm:2 ↔ CNS 3932 M 3 x 5:60
- Wstaw:79 [Insert]: Prowadnica liniowa typu MGN12H 600mm:2 ↔ CNS 3932 M 3 x 5:61
- Wstaw:80 [Insert]: Prowadnica liniowa typu MGN12H 600mm:1 ↔ CNS 3932 M 3 x 5:62
- Wstaw:81 [Insert]: Prowadnica liniowa typu MGN12H 600mm:1 ↔ CNS 3932 M 3 x 5:63
- Wstaw:82 [Insert]: Prowadnica liniowa typu MGN12H 600mm:1 ↔ CNS 3932 M 3 x 5:64
- Wstaw:83 [Insert]: Prowadnica liniowa typu MGN12H 600mm:1 ↔ CNS 3932 M 3 x 5:65
- Wstaw:84 [Insert]: Prowadnica liniowa typu MGN12H 600mm:1 ↔ CNS 3932 M 3 x 5:66
- Wstaw:85 [Insert]: Prowadnica liniowa typu MGN12H 600mm:1 ↔ CNS 3932 M 3 x 5:67
- Wstaw:86 [Insert]: Prowadnica liniowa typu MGN12H 600mm:1 ↔ CNS 3932 M 3 x 5:68
- Wstaw:87 [Insert]: Prowadnica liniowa typu MGN12H 600mm:1 ↔ CNS 3932 M 3 x 5:69
- Wstaw:88 [Insert]: Prowadnica liniowa typu MGN12H 600mm:1 ↔ CNS 3932 M 3 x 5:70
- Wstaw:89 [Insert]: Prowadnica liniowa typu MGN12H 600mm:1 ↔ CNS 3932 M 3 x 5:71
- Wstaw:90 [Insert]: Prowadnica liniowa typu MGN12H 600mm:1 ↔ CNS 3932 M 3 x 5:72
- Wstaw:91 [Insert]: Prowadnica liniowa typu MGN12H 600mm:1 ↔ CNS 3932 M 3 x 5:73
- Wstaw:92 [Insert]: Prowadnica liniowa typu MGN12H 600mm:1 ↔ CNS 3932 M 3 x 5:74
- Wstaw:93 [Insert]: Prowadnica liniowa typu MGN12H 600mm:1 ↔ CNS 3932 M 3 x 5:75
- Wstaw:94 [Insert]: Prowadnica liniowa typu MGN12H 600mm:1 ↔ CNS 3932 M 3 x 5:76
- Wstaw:95 [Insert]: Prowadnica liniowa typu MGN12H 600mm:1 ↔ CNS 3932 M 3 x 5:77
- Wstaw:96 [Insert]: Prowadnica liniowa typu MGN12H 600mm:1 ↔ CNS 3932 M 3 x 5:78
- Wstaw:97 [Insert]: Prowadnica liniowa typu MGN12H 600mm:1 ↔ CNS 3932 M 3 x 5:79
- Wstaw:98 [Insert]: Prowadnica liniowa typu MGN12H 600mm:1 ↔ CNS 3932 M 3 x 5:80
- Wstaw:99 [Insert]: Prowadnica liniowa typu MGN12H 600mm:1 ↔ CNS 3932 M 3 x 5:81
- Wstaw:100 [Insert]: Prowadnica liniowa typu MGN12H 600mm:1 ↔ CNS 3932 M 3 x 5:82
- Wstaw:101 [Insert]: Prowadnica liniowa typu MGN12H 600mm:1 ↔ CNS 3932 M 3 x 5:83
- Wstaw:102 [Insert]: Prowadnica liniowa typu MGN12H 600mm:1 ↔ CNS 3932 M 3 x 5:84
- Zestawiający:70 [Mate]: Prowadnica liniowa typu MGN12H 600mm:2 ↔ Wózek MGN12H:1
- Zestawiający:71 [Mate]: Prowadnica liniowa typu MGN12H 600mm:2 ↔ Wózek MGN12H:1
- Zestawiający:72 [Mate]: Prowadnica liniowa typu MGN12H 600mm:1 ↔ Wózek MGN12H:2
- Zestawiający:73 [Mate]: Prowadnica liniowa typu MGN12H 600mm:1 ↔ Wózek MGN12H:2
- Wstaw:103 [Insert]: Wspornik pionowy osi Z:1 ↔ CNS 3932 M 3 x 5:85
- Wstaw:104 [Insert]: Wspornik pionowy osi Z:1 ↔ CNS 3932 M 3 x 5:86
- Wstaw:105 [Insert]: Wspornik pionowy osi Z:1 ↔ CNS 3932 M 3 x 5:87
- Wstaw:106 [Insert]: Wspornik pionowy osi Z:1 ↔ CNS 3932 M 3 x 5:88
- Wstaw:107 [Insert]: Wspornik pionowy osi Z:1 ↔ CNS 3932 M 3 x 5:89
- Wstaw:108 [Insert]: Wspornik pionowy osi Z:1 ↔ CNS 3932 M 3 x 5:90
- Wstaw:109 [Insert]: Wspornik pionowy osi Z:1 ↔ CNS 3932 M 3 x 5:91
- Wstaw:110 [Insert]: Wspornik pionowy osi Z:1 ↔ CNS 3932 M 3 x 5:92
- Zestawiający:74 [Mate]: Wózek MGN12H:1 ↔ Wspornik pionowy osi Z:1
- Zestawiający:75 [Mate]: Wózek MGN12H:2 ↔ Wspornik pionowy osi Z:1
- Równoległy:56 [Flush]: Wózek MGN12H:1 ↔ Wózek MGN12H:2
- Zestawiający:76 [Mate]: Wózek MGN12H:1 ↔ Wspornik pionowy osi Z:1
- Zestawiający:77 [Mate]: Profil dolny posuwu osi Y:1 ↔ Wspornik pionowy osi Y - lewa strona:1
- Równoległy:57 [Flush]: Profil dolny posuwu osi Y:1 ↔ Wspornik pionowy osi Y - lewa strona:1
- Równoległy:58 [Flush]: Profil dolny posuwu osi Y:1 ↔ Wspornik pionowy osi Y - lewa strona:1
- Zestawiający:78 [Mate]: Łożysko kulowe jednorzędowe 6200 2RS:1 ↔ Wspornik pionowy osi Y - lewa strona:1
- Równoległy:59 [Flush]: Łożysko kulowe jednorzędowe 6200 2RS:1 ↔ Wspornik pionowy osi Y - lewa strona:1
- Zestawiający:79 [Mate]: Profil dolny posuwu osi Y:1 ↔ Wspornik pionowy osi Y - prawa strona:1
- Równoległy:60 [Flush]: Profil dolny posuwu osi Y:1 ↔ Wspornik pionowy osi Y - prawa strona:1
- Równoległy:61 [Flush]: Profil dolny posuwu osi Y:1 ↔ Wspornik pionowy osi Y - prawa strona:1
- Równoległy:63 [Flush]: Profil aluminiowy alutec K&K 104080:1 ↔ Prowadnica liniowa typu MGN12H 600mm:2
- Równoległy:64 [Flush]: Profil aluminiowy alutec K&K 104080:1 ↔ Prowadnica liniowa typu MGN12H 600mm:1
- Zestawiający:80 [Mate]: Wózek MGN9C:1 ↔ Wspornik pionowy osi Y - lewa strona:1
- Zestawiający:81 [Mate]: Wózek MGN9C:2 ↔ Wspornik pionowy osi Y - lewa strona:1
- Zestawiający:82 [Mate]: Wózek MGN9C:3 ↔ Wspornik pionowy osi Y - prawa strona:1
- Zestawiający:83 [Mate]: Wózek MGN9C:4 ↔ Wspornik pionowy osi Y - prawa strona:1
- Zestawiający:84 [Mate]: Profil aluminiowy alutec K&K 104080:1 ↔ Wspornik pionowy osi Y - prawa strona:1
- Równoległy:65 [Flush] (70 mm): Profil aluminiowy alutec K&K 104080:1 ↔ Wspornik pionowy osi Y - prawa strona:1
- Równoległy:66 [Flush]: Profil aluminiowy alutec K&K 104080:1 ↔ Wspornik pionowy osi Y - prawa strona:1
- Zestawiający:87 [Mate]: Łożysko kulowe jednorzędowe 3200 2RS:1 ↔ Śruba trapezowa 16x4 - oś X:1
- Zestawiający:88 [Mate]: Łożysko kulowe jednorzędowe 3200 2RS:1 ↔ Śruba trapezowa 16x4 - oś X:1
- Zestawiający:89 [Mate]: Śruba trapezowa 16x4 - oś X:1 ↔ DIN 6926 - zastąpiona przez DIN EN 1663/1666 M10:2
- Zestawiający:90 [Mate]: Łożysko kulowe jednorzędowe 3200 2RS:1 ↔ DIN 6926 - zastąpiona przez DIN EN 1663/1666 M10:2
- Zestawiający:94 [Mate] (70 mm): Wrzeciono Elektrowrzeciono CNC 0.8kw:1 ↔ Sklejka stołu:1
- Zestawiający:96 [Mate]: Wspornik pionowy osi Y - prawa strona:1 ↔ Łożysko kulowe jednorzędowe 3200 2RS:1
- Równoległy:67 [Flush]: Wspornik pionowy osi Y - prawa strona:1 ↔ Wspornik łożyska osi Y - prawa strona:1
- Zestawiający:97 [Mate]: Wspornik pionowy osi Y - prawa strona:1 ↔ Wspornik łożyska osi Y - prawa strona:1
- Równoległy:68 [Flush]: Wspornik pionowy osi Y - prawa strona:1 ↔ Wspornik łożyska osi Y - prawa strona:1
- Zestawiający:98 [Mate]: Wspornik łożyska osi Y - prawa strona:1 ↔ CNS 3932 M 3 x 14:2
- Zestawiający:99 [Mate]: Wspornik łożyska osi Y - prawa strona:1 ↔ CNS 3932 M 3 x 14:2
- Zestawiający:100 [Mate]: Wspornik łożyska osi Y - prawa strona:1 ↔ CNS 3932 M 3 x 14:3
- Zestawiający:101 [Mate]: Wspornik łożyska osi Y - prawa strona:1 ↔ CNS 3932 M 3 x 14:3
- Zestawiający:102 [Mate]: Wspornik łożyska osi Y - prawa strona:1 ↔ CNS 3932 M 3 x 14:1
- Zestawiający:103 [Mate]: Wspornik łożyska osi Y - prawa strona:1 ↔ CNS 3932 M 3 x 14:1
- Zestawiający:104 [Mate]: Wspornik łożyska osi Y - prawa strona:1 ↔ CNS 3932 M 3 x 14:4
- Zestawiający:105 [Mate]: Wspornik łożyska osi Y - prawa strona:1 ↔ CNS 3932 M 3 x 14:4
- Zestawiający:106 [Mate]: Wspornik pionowy osi Z:1 ↔ Obudowa nakrętki trapezowej fi 16:2
- Zestawiający:107 [Mate]: Wspornik pionowy osi Z:1 ↔ Obudowa nakrętki trapezowej fi 16:2
- Zestawiający:108 [Mate]: Wspornik pionowy osi Z:1 ↔ Obudowa nakrętki trapezowej fi 16:2
- Zestawiający:109 [Mate]: Nakrętka trapezowa kołnierzowa JFRM-2835TR16x4:2 ↔ Obudowa nakrętki trapezowej fi 16:2
- Zestawiający:110 [Mate]: Nakrętka trapezowa kołnierzowa JFRM-2835TR16x4:2 ↔ Obudowa nakrętki trapezowej fi 16:2
- Zestawiający:111 [Mate]: Nakrętka trapezowa kołnierzowa JFRM-2835TR16x4:2 ↔ Obudowa nakrętki trapezowej fi 16:2
- Zestawiający:112 [Mate]: Nakrętka trapezowa kołnierzowa JFRM-2835TR16x4:1 ↔ Obudowa nakrętki trapezowej fi 16:1
- Zestawiający:113 [Mate]: Nakrętka trapezowa kołnierzowa JFRM-2835TR16x4:1 ↔ Obudowa nakrętki trapezowej fi 16:1
- Wstaw:111 [Insert]: Nakrętka trapezowa kołnierzowa JFRM-2835TR16x4:2 ↔ CNS 3932 M 5 x 10:9
- Wstaw:112 [Insert]: Nakrętka trapezowa kołnierzowa JFRM-2835TR16x4:2 ↔ CNS 3932 M 5 x 10:10
- Wstaw:113 [Insert]: Nakrętka trapezowa kołnierzowa JFRM-2835TR16x4:2 ↔ CNS 3932 M 5 x 10:11
- Wstaw:114 [Insert]: Nakrętka trapezowa kołnierzowa JFRM-2835TR16x4:2 ↔ CNS 3932 M 5 x 10:12
- Wstaw:115 [Insert]: Nakrętka trapezowa kołnierzowa JFRM-2835TR16x4:2 ↔ CNS 3932 M 5 x 10:13
- Wstaw:116 [Insert]: Nakrętka trapezowa kołnierzowa JFRM-2835TR16x4:2 ↔ CNS 3932 M 5 x 10:14
- Wstaw:117 [Insert]: Nakrętka trapezowa kołnierzowa JFRM-2835TR16x4:1 ↔ CNS 3932 M 5 x 10:15
- Wstaw:118 [Insert]: Nakrętka trapezowa kołnierzowa JFRM-2835TR16x4:1 ↔ CNS 3932 M 5 x 10:16
- Wstaw:119 [Insert]: Nakrętka trapezowa kołnierzowa JFRM-2835TR16x4:1 ↔ CNS 3932 M 5 x 10:17
- Wstaw:120 [Insert]: Nakrętka trapezowa kołnierzowa JFRM-2835TR16x4:1 ↔ CNS 3932 M 5 x 10:18
- Wstaw:121 [Insert]: Nakrętka trapezowa kołnierzowa JFRM-2835TR16x4:1 ↔ CNS 3932 M 5 x 10:19
- Wstaw:122 [Insert]: Nakrętka trapezowa kołnierzowa JFRM-2835TR16x4:1 ↔ CNS 3932 M 5 x 10:20
- Wstaw:123 [Insert]: Obudowa nakrętki trapezowej fi 16:2 ↔ CNS 3932 M 5 x 12:5
- Wstaw:124 [Insert]: Obudowa nakrętki trapezowej fi 16:2 ↔ CNS 3932 M 5 x 12:8
- Wstaw:125 [Insert]: Obudowa nakrętki trapezowej fi 16:2 ↔ CNS 3932 M 5 x 12:6
- Wstaw:126 [Insert]: Obudowa nakrętki trapezowej fi 16:2 ↔ CNS 3932 M 5 x 12:7
- Równoległy:69 [Flush]: Wspornik pionowy osi Y - prawa strona:1 ↔ Łożysko kulowe jednorzędowe 3200 2RS:1
- Zestawiający:114 [Mate]: Koło zębate 21 T5 28 2F:2 ↔ Tuleja zaciskowo rozprężna RCK BK 80 8x15 Clampex:2
- Zestawiający:115 [Mate]: Koło zębate 21 T5 28 2F:2 ↔ Tuleja zaciskowo rozprężna RCK BK 80 8x15 Clampex:2
- Zestawiający:116 [Mate]: Śruba trapezowa 16x4 - oś X:1 ↔ Tuleja zaciskowo rozprężna RCK BK 80 8x15 Clampex:2
- Wstaw:127 [Insert]: Tuleja zaciskowo rozprężna RCK BK 80 8x15 Clampex:2 ↔ CNS 3932 M 4 x 6:7
- Wstaw:128 [Insert]: Tuleja zaciskowo rozprężna RCK BK 80 8x15 Clampex:2 ↔ CNS 3932 M 4 x 6:8
- Wstaw:129 [Insert]: Tuleja zaciskowo rozprężna RCK BK 80 8x15 Clampex:2 ↔ CNS 3932 M 4 x 6:9
- Wstaw:130 [Insert]: Tuleja zaciskowo rozprężna RCK BK 80 8x15 Clampex:2 ↔ CNS 3932 M 4 x 6:10
- Wstaw:131 [Insert]: Tuleja zaciskowo rozprężna RCK BK 80 8x15 Clampex:2 ↔ CNS 3932 M 4 x 6:11
- Wstaw:132 [Insert]: Tuleja zaciskowo rozprężna RCK BK 80 8x15 Clampex:2 ↔ CNS 3932 M 4 x 6:12
- Zestawiający:117 [Mate] (2 mm): Śruba trapezowa 16x4 - oś X:1 ↔ Tuleja zaciskowo rozprężna RCK BK 80 8x15 Clampex:2
- Zestawiający:118 [Mate]: Silnik krokowy SM 60 100-4004AF - 4Nm:2 ↔ Koło zębate 21 T5 14 2F:2
- Zestawiający:119 [Mate] (1 mm): Silnik krokowy SM 60 100-4004AF - 4Nm:2 ↔ Koło zębate 21 T5 14 2F:2
- Zestawiający:120 [Mate] (18 mm): Wspornik pionowy osi Y - prawa strona:1 ↔ Silnik krokowy SM 60 100-4004AF - 4Nm:2
- Równoległy:70 [Flush]: Koło zębate 21 T5 28 2F:2 ↔ Koło zębate 21 T5 14 2F:2
- Zestawiający:123 [Mate]: Silnik krokowy SM 60 100-4004AF - 4Nm:2 ↔ Uchwyt silnika krokowego osi X:1
- Zestawiający:124 [Mate]: Silnik krokowy SM 60 100-4004AF - 4Nm:2 ↔ Uchwyt silnika krokowego osi X:1
- Zestawiający:125 [Mate]: Silnik krokowy SM 60 100-4004AF - 4Nm:2 ↔ Uchwyt silnika krokowego osi X:1
- Wstaw:133 [Insert]: Wspornik pionowy osi Y - lewa strona:1 ↔ CNS 3932 M 8 x 14:1
- Wstaw:134 [Insert]: Wspornik pionowy osi Y - lewa strona:1 ↔ CNS 3932 M 8 x 14:2
- Wstaw:135 [Insert]: Wspornik pionowy osi Y - prawa strona:1 ↔ CNS 3932 M 8 x 14:3
- Wstaw:136 [Insert]: Wspornik pionowy osi Y - prawa strona:1 ↔ CNS 3932 M 8 x 14:4
- Zestawiający:129 [Mate]: Koło zębate 21 T5 28 2F:2 ↔ Pas zębaty 10 T5-295:1
- Zestawiający:130 [Mate]: Koło zębate 21 T5 14 2F:2 ↔ Pas zębaty 10 T5-295:1
- Zestawiający:131 [Mate]: Koło zębate 21 T5 14 2F:2 ↔ Pas zębaty 10 T5-295:1
- Zestawiający:135 [Mate]: Profil dolny długi:2 ↔ Profil dolny krótki:2
- Zestawiający:136 [Mate]: Koło zębate 21 T5 28 2F:1 ↔ Pas zębaty 10 T5-295:2
- Zestawiający:137 [Mate]: Koło zębate 21 T5 14 2F:1 ↔ Pas zębaty 10 T5-295:2
- Zestawiający:138 [Mate]: Koło zębate 21 T5 14 2F:1 ↔ Pas zębaty 10 T5-295:2
- Wstaw:145 [Insert]: Wspornik pionowy osi Y - prawa strona:1 ↔ CNS 3932 M 4 x 6:21
- Wstaw:146 [Insert]: Wspornik pionowy osi Y - prawa strona:1 ↔ CNS 3932 M 4 x 6:22
- Wstaw:147 [Insert]: Wspornik pionowy osi Y - prawa strona:1 ↔ CNS 3932 M 4 x 6:23
- Wstaw:148 [Insert]: Wspornik pionowy osi Y - prawa strona:1 ↔ CNS 3932 M 4 x 6:24
- Wstaw:149 [Insert]: Wspornik pionowy osi Y - prawa strona:1 ↔ CNS 3932 M 4 x 6:25
- Wstaw:150 [Insert]: Wspornik pionowy osi Y - prawa strona:1 ↔ CNS 3932 M 4 x 6:26
- Wstaw:151 [Insert]: Wspornik pionowy osi Y - prawa strona:1 ↔ CNS 3932 M 4 x 6:27
- Wstaw:152 [Insert]: Wspornik pionowy osi Y - prawa strona:1 ↔ CNS 3932 M 4 x 6:28
- Zestawiający:139 [Mate]: Wspornik pionowy osi Y - prawa strona:1 ↔ CNS 3932 M 4 x 16:1
- Zestawiający:140 [Mate]: Uchwyt silnika krokowego osi X:1 ↔ CNS 3932 M 4 x 16:1
- Zestawiający:141 [Mate]: Wspornik pionowy osi Y - prawa strona:1 ↔ CNS 3932 M 4 x 16:2
- Zestawiający:142 [Mate]: Uchwyt silnika krokowego osi X:1 ↔ CNS 3932 M 4 x 16:2
- Zestawiający:143 [Mate]: Wspornik pionowy osi Y - prawa strona:1 ↔ CNS 3932 M 4 x 16:3
- Zestawiający:144 [Mate]: Uchwyt silnika krokowego osi X:1 ↔ CNS 3932 M 4 x 16:3
- Zestawiający:145 [Mate]: Wspornik pionowy osi Y - prawa strona:1 ↔ CNS 3932 M 4 x 16:4
- Zestawiający:146 [Mate]: Uchwyt silnika krokowego osi X:1 ↔ CNS 3932 M 4 x 16:4
- Wstaw:153 [Insert]: Silnik krokowy SM 60 100-4004AF - 4Nm:2 ↔ CNS 3932 M 5 x 12:10
- Wstaw:154 [Insert]: Silnik krokowy SM 60 100-4004AF - 4Nm:2 ↔ CNS 3932 M 5 x 12:11
- Wstaw:155 [Insert]: Silnik krokowy SM 60 100-4004AF - 4Nm:2 ↔ CNS 3932 M 5 x 12:12
- Wstaw:156 [Insert]: Silnik krokowy SM 60 100-4004AF - 4Nm:2 ↔ CNS 3932 M 5 x 12:13
